# Autodesk Inventor assembly: Сборка1
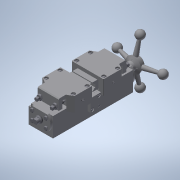
[picture p0: Inventor's stored thumbnail of the model, 180x180]
Saved by Autodesk Inventor 2022 (Build 260153000, 153)
## iProperties
Created: 2014-04-12
Part Number: Сборка1
Document SubType Name: Assembly
Designer: Украинцев
Mass: 3956.86 g
Surface Area: 5400.32 cm^2
Volume: 2783.85 cm^3
Density: 1.42136 g/cm^3
Author: Украинцев
## Documents named in this file (23)
- C:\Users\сервер\Desktop\Новая папка (5)\Workspace\Тиски.iam
- C:\Users\сервер\Desktop\Новая папка (5)\Workspace\Угольник 10.ipt
- C:\Users\сервер\Desktop\Новая папка (5)\Workspace\Колонка 1.ipt
- C:\Users\сервер\Desktop\Новая папка (5)\Workspace\Губка 2.ipt
- C:\Users\сервер\Desktop\Новая папка (5)\Workspace\Втулка 12.ipt
- C:\Users\сервер\Desktop\Новая папка (5)\Workspace\Втулка 4.ipt
- C:\Users\сервер\Desktop\Новая папка (5)\Workspace\Сборка1\Мастер проектирования\Винт 3.iam
- C:\Users\сервер\Desktop\Новая папка (5)\Workspace\Фиксатор 11.ipt
- C:\Users\сервер\Desktop\Новая папка (5)\Workspace\Призма 5.ipt
- C:\Users\сервер\Desktop\Новая папка (5)\Workspace\Крышка 6.ipt
- C:\Users\сервер\Desktop\Новая папка (5)\Workspace\Гайка 7.ipt
- C:\Users\сервер\Desktop\Новая папка (5)\Workspace\Рукоятка 8.ipt
- C:\Users\сервер\Desktop\Новая папка (5)\Workspace\Ручка 9.ipt
- C:\Users\сервер\Desktop\Новая папка (5)\Libraries\Content Center Files\ru-RU\GOST 7808-70\Болт M10-6gx30 ГОСТ 7808-70.ipt
- C:\Users\сервер\Desktop\Новая папка (5)\Libraries\Content Center Files\ru-RU\GOST 7808-70\Болт M16-6gx45 ГОСТ 7808-70.ipt
- C:\Users\сервер\Desktop\Новая папка (5)\Libraries\Content Center Files\ru-RU\GOST 7808-70\Болт M8-6gx20 ГОСТ 7808-70.ipt
- C:\Users\сервер\Desktop\Новая папка (5)\Libraries\Content Center Files\ru-RU\GOST 1491-80 A\Винт M8-6gx12 ГОСТ 1491-80.ipt
- C:\Users\сервер\Desktop\Новая папка (5)\Libraries\Content Center Files\ru-RU\GOST 5916-70\Гайка M10-6H ГОСТ 5916-70.ipt
- C:\Users\сервер\Desktop\Новая папка (5)\Libraries\Content Center Files\ru-RU\GOST 1482-84\Винт M10-6gx40 ГОСТ 1482-84.ipt
- C:\Users\сервер\Desktop\Новая папка (5)\Libraries\Content Center Files\ru-RU\Screw GOST 1477-93\Винт M8-6gx25 ГОСТ 1477-93.ipt
- C:\Users\сервер\Desktop\Новая папка (5)\Libraries\Content Center Files\ru-RU\GOST 3128-70 (2)\Штифт 2.3x20 ГОСТ 3128-70.ipt
- C:\Users\сервер\Desktop\Новая папка (5)\Libraries\Content Center Files\ru-RU\GOST 3128-70 (2)\Штифт 2.8x30 ГОСТ 3128-70.ipt
- C:\Users\сервер\Desktop\Новая папка (5)\Libraries\Content Center Files\ru-RU\GOST 3128-70 (2)\Штифт 2.5x30 ГОСТ 3128-70.ipt
## Components (57 placed, 22 different names)
1. Болт M10-6gx30 ГОСТ 7808-70.ipt:14
2. Болт M16-6gx45 ГОСТ 7808-70.ipt:15
3. Винт 3.iam:16 [sub-assembly] — Вращательный:1, РеечПер:1, РеечПер:2, Жесткий:10, Угол:1
4. Винт M8-6gx12 ГОСТ 1491-80.ipt:1
5. Винт M8-6gx12 ГОСТ 1491-80.ipt:2
6. Винт ГОСТ 1477-93 M8x25-B:1
7. Винт ГОСТ 1477-93 M8x25-B:2
8. Втулка 12.ipt:3 — Жесткий:3, РеечПер:1, Угол:1
9. Втулка 4.ipt:4 — Жесткий:4, РеечПер:2
10. Гайка 7.ipt:5 — Жесткий:10, Совмещение:1, Совмещение:2
11. Губка 2.ipt:6 — Плоский:1, Цилиндрический:1, Жесткий:3, Жесткий:6, Жесткий:8
12. Губка 2.ipt:7 — Плоский:2, Цилиндрический:2, Жесткий:4, Жесткий:7, Жесткий:9
13. Колонка 1.ipt:8 — Жесткий:1, Цилиндрический:1, Цилиндрический:2, Вращательный:1, Жесткий:5
14. Крышка 6.ipt:10 — Жесткий:9
15. Крышка 6.ipt:9 — Жесткий:8
16. Призма 5.ipt:11 — Жесткий:6
17. Призма 5.ipt:12 — Жесткий:7
18. Угольник 10.ipt:13 — Жесткий:1, Плоский:1, Плоский:2
19. Фиксатор 11.ipt:17 — Жесткий:5
20. Штифты 2 ГОСТ 3128-70 8 x  30:1
21. Штифты 2 ГОСТ 3128-70 5 x  30:1
22. Штифты 2 ГОСТ 3128-70 3 x  20:1
23. Штифты 2 ГОСТ 3128-70 3 x  20:2
24. Штифты 2 ГОСТ 3128-70 3 x  20:3
25. Штифты 2 ГОСТ 3128-70 3 x  20:4
26. Рукоятка 8.ipt:18 — Жесткий:12, Совмещение:1, Совмещение:2
27. Ручка 9.ipt:19 — Жесткий:12
28. Рукоятка 8.ipt:20
29. Ручка 9.ipt:21
30. Рукоятка 8.ipt:22
31. Ручка 9.ipt:23
32. Рукоятка 8.ipt:24
33. Ручка 9.ipt:25
34. Болт M8-6gx20 ГОСТ 7808-70.ipt:26
35. Болт M8-6gx20 ГОСТ 7808-70.ipt:27
36. Болт M8-6gx20 ГОСТ 7808-70.ipt:28
37. Болт M8-6gx20 ГОСТ 7808-70.ipt:29
38. Болт M8-6gx20 ГОСТ 7808-70.ipt:30
39. Болт M8-6gx20 ГОСТ 7808-70.ipt:31
40. Болт M8-6gx20 ГОСТ 7808-70.ipt:32
41. Болт M8-6gx20 ГОСТ 7808-70.ipt:33
42. Винт M8-6gx12 ГОСТ 1491-80.ipt:34
43. Винт M8-6gx12 ГОСТ 1491-80.ipt:35
44. Винт M8-6gx12 ГОСТ 1491-80.ipt:36
45. Винт M8-6gx12 ГОСТ 1491-80.ipt:37
46. Винт M8-6gx12 ГОСТ 1491-80.ipt:39
47. Винт M8-6gx12 ГОСТ 1491-80.ipt:40
48. Винт M8-6gx12 ГОСТ 1491-80.ipt:41
49. Винт M8-6gx12 ГОСТ 1491-80.ipt:42
50. Гайка ГОСТ 5916-70 M10:1
51. Винт ГОСТ 1482-84 M 10 x 40:1
52. Гайка ГОСТ 5916-70 M10:3
53. Винт ГОСТ 1482-84 M 10 x 40:3
54. Винт ГОСТ 1482-84 M 10 x 40:2
55. Гайка ГОСТ 5916-70 M10:2
56. Винт ГОСТ 1482-84 M 10 x 40:4
57. Гайка ГОСТ 5916-70 M10:4
## Component patterns: (4 elements, first: Штифты 2 ГОСТ 3128-70 3 x  20:1), (4 elements, first: Рукоятка 8.ipt:18 + Ручка 9.ipt:19), (4 elements, first: Болт M8-6gx20 ГОСТ 7808-70.ipt:26), МассивКомп 3:1 (4 elements), МассивКомп 4:1 (4 elements), МассивКомп 5:1 (4 elements), МассивКомп 6:1 (2 elements), МассивКомп 7:1 (2 elements)
## Relationships (20: WeldJoint 10, PlanarJoint 2, CylindricalJoint 2, RelateRotateTranslate 2, Mate 2, RevoluteJoint 1, Angle 1)
- Жесткий:1 [WeldJoint]: Колонка 1.ipt:8 ↔ Угольник 10.ipt:13
- Плоский:1 [PlanarJoint]: Губка 2.ipt:6 ↔ Угольник 10.ipt:13
- Цилиндрический:1 [CylindricalJoint]: Губка 2.ipt:6 ↔ Колонка 1.ipt:8
- Плоский:2 [PlanarJoint]: Губка 2.ipt:7 ↔ Угольник 10.ipt:13
- Цилиндрический:2 [CylindricalJoint]: Губка 2.ipt:7 ↔ Колонка 1.ipt:8
- Жесткий:3 [WeldJoint]: Втулка 12.ipt:3 ↔ Губка 2.ipt:6
- Жесткий:4 [WeldJoint]: Втулка 4.ipt:4 ↔ Губка 2.ipt:7
- Вращательный:1 [RevoluteJoint]: Винт 3.iam:16 ↔ Колонка 1.ipt:8
- РеечПер:1 [RelateRotateTranslate] (5 mm): Винт 3.iam:16 ↔ Втулка 12.ipt:3
- РеечПер:2 [RelateRotateTranslate] (5 mm): Винт 3.iam:16 ↔ Втулка 4.ipt:4
- Жесткий:5 [WeldJoint]: Колонка 1.ipt:8 ↔ Фиксатор 11.ipt:17
- Жесткий:6 [WeldJoint] (18.5 mm): Губка 2.ipt:6 ↔ Призма 5.ipt:11
- Жесткий:7 [WeldJoint] (18.5 mm): Губка 2.ipt:7 ↔ Призма 5.ipt:12
- Жесткий:8 [WeldJoint]: Губка 2.ipt:6 ↔ Крышка 6.ipt:9
- Жесткий:9 [WeldJoint]: Губка 2.ipt:7 ↔ Крышка 6.ipt:10
- Жесткий:10 [WeldJoint]: Винт 3.iam:16 ↔ Гайка 7.ipt:5
- Жесткий:12 [WeldJoint]: Рукоятка 8.ipt:18 ↔ Ручка 9.ipt:19
- Совмещение:1 [Mate]: Гайка 7.ipt:5 ↔ Рукоятка 8.ipt:18
- Совмещение:2 [Mate]: Гайка 7.ipt:5 ↔ Рукоятка 8.ipt:18
- Угол:1 [Angle] (0 deg): Винт 3.iam:16 ↔ Втулка 12.ipt:3
